# Autodesk Inventor assembly: 組合1(更)
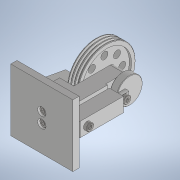
[picture p0: Inventor's stored thumbnail of the model, 180x180]
Saved by Autodesk Inventor 2020 (Build 240168000, 168)
## iProperties
Created: 2021-03-15
Part Number: 組合1(更)
Document SubType Name: Assembly
Designer: Sugar
Author: Sugar
## Documents named in this file (10)
- E:\github\cd2021\零件圖\組合1(更).iam
- E:\github\cd2021\零件圖\零件3.ipt
- E:\github\cd2021\零件圖\零件1.ipt
- E:\github\cd2021\零件圖\零件2.ipt
- E:\github\cd2021\零件圖\零件4.ipt
- E:\github\cd2021\零件圖\零件5(更).ipt
- E:\github\cd2021\零件圖\零件6(更).ipt
- E:\github\cd2021\零件圖\零件7(更).ipt
- E:\github\cd2021\零件圖\DIN 6912 - M5 x 10.ipt
- E:\github\cd2021\零件圖\DIN 6912 - M5 x 12.ipt
## Components (16 placed, 9 different names)
1. 零件3:1 — 插入:1, 插入:2, 貼合:35, 貼合:36, 角度:1
2. 零件1:1 — 插入:1, 插入:2, 插入:3, 插入:4, 貼合:8, 貼合:14, 貼合:33, 貼合:34
3. 零件2:2 — 插入:4, 貼合:4, 插入:8
4. 零件2:4 — 插入:3, 貼合:3, 插入:7
5. 零件4:1 — 貼合:2, 貼合:21, 插入:6
6. 零件4:2 — 貼合:1, 貼合:24, 插入:5
7. 零件5(更):1 — 貼合:7, 貼合:10, 貼合:12, 貼合:15, 貼合:18, 貼合:26, 角度:1
8. 零件6(更):1 — 貼合:10, 貼合:11, 貼合:14, 貼合:15, 貼合:16, 貼合:23, 貼合:27
9. 零件7(更):1 — 貼合:16, 貼合:17, 貼合:20, 貼合:26, 貼合:29
10. DIN 6912 - M5 x 10:1 — 貼合:28, 貼合:29
11. DIN 6912 - M5 x 10:5 — 貼合:31, 貼合:36
12. DIN 6912 - M5 x 10:6 — 貼合:32, 貼合:35
13. DIN 6912 - M5 x 10:7 — 插入:6
14. DIN 6912 - M5 x 10:8 — 插入:5
15. DIN 6912 - M5 x 12:1 — 插入:7
16. DIN 6912 - M5 x 12:2 — 插入:8
## Relationships (47: Mate 38, Insert 8, Angle 1)
- 插入:1 [Insert]: 零件3:1 ↔ 零件1:1
- 插入:2 [Insert]: 零件3:1 ↔ 零件1:1
- 插入:3 [Insert]: 零件1:1 ↔ 零件2:4
- 插入:4 [Insert]: 零件1:1 ↔ 零件2:2
- 貼合:1 [Mate]: 零件4:2
- 貼合:2 [Mate]: 零件4:1
- 貼合:3 [Mate]: 零件2:4
- 貼合:4 [Mate]: 零件2:2
- 貼合:5 [Mate]
- 貼合:6 [Mate]
- 貼合:7 [Mate]: 零件5(更):1
- 貼合:8 [Mate]: 零件1:1
- 貼合:9 [Mate]
- 貼合:10 [Mate]: 零件5(更):1 ↔ 零件6(更):1
- 貼合:11 [Mate]: 零件6(更):1
- 貼合:12 [Mate]: 零件5(更):1
- 貼合:13 [Mate]
- 貼合:14 [Mate]: 零件1:1 ↔ 零件6(更):1
- 貼合:15 [Mate]: 零件5(更):1 ↔ 零件6(更):1
- 貼合:16 [Mate]: 零件6(更):1 ↔ 零件7(更):1
- 貼合:17 [Mate]: 零件7(更):1
- 貼合:18 [Mate]: 零件5(更):1
- 貼合:19 [Mate]
- 貼合:20 [Mate]: 零件7(更):1
- 貼合:21 [Mate]: 零件4:1
- 貼合:22 [Mate]
- 貼合:23 [Mate]: 零件6(更):1
- 貼合:24 [Mate]: 零件4:2
- 貼合:25 [Mate]
- 貼合:26 [Mate]: 零件5(更):1 ↔ 零件7(更):1
- 貼合:27 [Mate]: 零件6(更):1
- 貼合:28 [Mate]: DIN 6912 - M5 x 10:1
- 貼合:29 [Mate]: 零件7(更):1 ↔ DIN 6912 - M5 x 10:1
- 貼合:30 [Mate]
- 貼合:31 [Mate]: DIN 6912 - M5 x 10:5
- 貼合:32 [Mate]: DIN 6912 - M5 x 10:6
- 貼合:33 [Mate]: 零件1:1
- 貼合:34 [Mate]: 零件1:1
- 貼合:35 [Mate]: 零件3:1 ↔ DIN 6912 - M5 x 10:6
- 貼合:36 [Mate]: 零件3:1 ↔ DIN 6912 - M5 x 10:5
- 貼合:37 [Mate]
- 貼合:38 [Mate]
- 插入:5 [Insert]: 零件4:2 ↔ DIN 6912 - M5 x 10:8
- 插入:6 [Insert]: 零件4:1 ↔ DIN 6912 - M5 x 10:7
- 插入:7 [Insert]: 零件2:4 ↔ DIN 6912 - M5 x 12:1
- 插入:8 [Insert]: 零件2:2 ↔ DIN 6912 - M5 x 12:2
- 角度:1 [Angle] (0 deg): 零件3:1 ↔ 零件5(更):1
